# Autodesk Inventor assembly: Assembly1
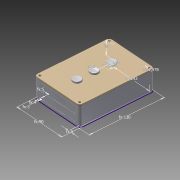
[picture p0: Inventor's stored thumbnail of the model, 180x180]
Saved by Autodesk Inventor 2013 (Build 170138000, 138)
## iProperties
Created: 2013-01-11
Part Number: Assembly1
Document SubType Name: Assembly
Designer: md
Author: md
## Documents named in this file (5)
- X:\Projects\hexasense\enclosure\sense_board\Assembly1.iam
- X:\Projects\hexasense\enclosure\sense_board\frontplatte.ipt
- X:\Projects\hexasense\enclosure\sense_board\pushbutton.ipt
- X:\Projects\hexasense\enclosure\sense_board\PCB-Model.ipt
- X:\Projects\hexasense\enclosure\sense_board\base.ipt
## Components (6 placed, 4 different names)
1. frontplatte:1 — Insert:6, Insert:7, Mate:1
2. pushbutton:1 — Insert:2
3. pushbutton:2 — Insert:3
4. pushbutton:3 — Insert:1
5. PCB-Model:1 — Insert:1, Insert:2, Insert:3
6. base:1 — Insert:6, Insert:7, Mate:1
## Relationships (6: Insert 5, Mate 1)
- Insert:1 (-5 mm): pushbutton:3 ↔ PCB-Model:1
- Insert:2 (-5 mm): pushbutton:1 ↔ PCB-Model:1
- Insert:3 (-5 mm): pushbutton:2 ↔ PCB-Model:1
- Insert:6: frontplatte:1 ↔ base:1
- Insert:7: frontplatte:1 ↔ base:1
- Mate:1: frontplatte:1 ↔ base:1
